# Autodesk Inventor assembly: Extruder
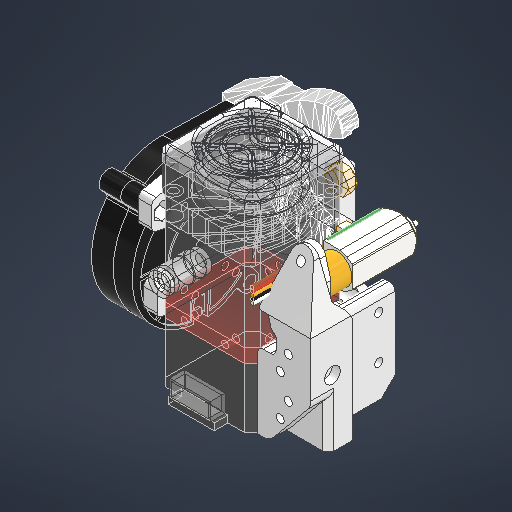
[picture p0: Inventor's stored thumbnail of the model, 512x512]
Saved by Autodesk Inventor 2026.2 (Build 302298000, 298)
## iProperties
Created: 2026-03-27
Part Number: Extruder
Document SubType Name: Assembly
Designer: gaoet
Author: gaoet
## Documents named in this file (7)
- C:\Users\gaoet\OneDrive\Desktop\Scissor 3D Printer\Extruder.iam
- C:\Users\gaoet\OneDrive\Desktop\Scissor 3D Printer\Hotend\Hotend\Hotend.ipt
- C:\Users\gaoet\OneDrive\Desktop\Scissor 3D Printer\Hotend\Fan_Duct.ipt
- C:\Users\gaoet\OneDrive\Desktop\Scissor 3D Printer\Radial-Cooling-Fan-5015-DC12V\Radial-Cooling-Fan-5015-DC12V\Radial-Cooling-Fan-5015-DC12V.ipt
- C:\Users\gaoet\OneDrive\Desktop\Scissor 3D Printer\BLTouch-Smart V3.1\BLTouch-Smart V3.1\BLTouch-Smart V3.1.ipt
- C:\Users\gaoet\OneDrive\Desktop\Scissor 3D Printer\ExtruderMount.ipt
- C:\Users\gaoet\OneDrive\Desktop\Scissor 3D Printer\FanMountV2.ipt
## Components (6 placed, 6 different names)
1. Hotend:1 — Insert:7, Mate:1, Insert:10, Insert:11
2. Fan_Duct:1 — Angle:2, Insert:12, Mate:4
3. Radial-Cooling-Fan-5015-DC12V:1 — Angle:2, Mate:2, Mate:3, Mate:4
4. ExtruderMount:1 — Insert:7, Mate:1, Insert:8, Insert:9
5. BLTouch-Smart V3.1:1 — Insert:8, Insert:9
6. FanMountV2:1 — Insert:10, Insert:11, Insert:12, Mate:2, Mate:3
## Relationships (11: Insert 6, Mate 4, Angle 1)
- Angle:2 (180 deg): Fan_Duct:1 ↔ Radial-Cooling-Fan-5015-DC12V:1
- Insert:7: Hotend:1 ↔ ExtruderMount:1
- Mate:1: Hotend:1 ↔ ExtruderMount:1
- Insert:8: ExtruderMount:1 ↔ BLTouch-Smart V3.1:1
- Insert:9: ExtruderMount:1 ↔ BLTouch-Smart V3.1:1
- Insert:10: Hotend:1 ↔ FanMountV2:1
- Insert:11: Hotend:1 ↔ FanMountV2:1
- Insert:12: Fan_Duct:1 ↔ FanMountV2:1
- Mate:2: Radial-Cooling-Fan-5015-DC12V:1 ↔ FanMountV2:1
- Mate:3: Radial-Cooling-Fan-5015-DC12V:1 ↔ FanMountV2:1
- Mate:4: Fan_Duct:1 ↔ Radial-Cooling-Fan-5015-DC12V:1
